# Autodesk Inventor assembly: x_chain_angle
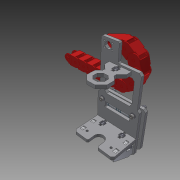
[picture p0: Inventor's stored thumbnail of the model, 180x180]
Saved by Autodesk Inventor 2014 (Build 180170000, 170)
## iProperties
Created: 2013-12-06
Part Number: x_chain_angle
Document SubType Name: Assembly
Designer: buben
Author: buben
## Documents named in this file (4)
- C:\Users\buben\Documents\GitHub\bacon\inventor files\assemblies\x_chain_angle.iam
- C:\Users\buben\Documents\GitHub\bacon\inventor files\assemblies\x_carryage.iam
- C:\Users\buben\Documents\GitHub\bacon\inventor files\utils\x_axis_cable_mount_b.ipt
- C:\Users\buben\Documents\GitHub\bacon\inventor files\utils\cable_chain_22.ipt
## Components (12 placed, 3 different names)
1. x_carryage:1 [sub-assembly] — Flush:1, Mate:1, Mate:2, Mate:3, Mate:4, Mate:5
2. x_axis_cable_mount_b:1 — Mate:3, Mate:4, Mate:5, Insert:10, Mate:6
3. cable_chain_22:1 — Insert:2, Insert:3, Mate:13, Mate:14
4. cable_chain_22:2 — Insert:4, Insert:5, Mate:11, Mate:12
5. cable_chain_22:3 — Insert:1, Mate:15
6. cable_chain_22:4 — Insert:1, Insert:2, Mate:14, Mate:15
7. cable_chain_22:5 — Insert:3, Insert:4, Mate:12, Mate:13
8. cable_chain_22:6 — Insert:5, Insert:6, Mate:10, Mate:11
9. cable_chain_22:7 — Insert:6, Insert:7, Mate:9, Mate:10
10. cable_chain_22:8 — Insert:7, Insert:8, Mate:8, Mate:9
11. cable_chain_22:9 — Insert:8, Insert:9, Mate:7, Mate:8
12. cable_chain_22:10 — Insert:9, Insert:10, Mate:6, Mate:7
## Relationships (26: Mate 15, Insert 10, Flush 1)
- Flush:1: x_carryage:1
- Mate:1: x_carryage:1
- Mate:2: x_carryage:1
- Mate:3: x_carryage:1 ↔ x_axis_cable_mount_b:1
- Mate:4: x_carryage:1 ↔ x_axis_cable_mount_b:1
- Mate:5: x_carryage:1 ↔ x_axis_cable_mount_b:1
- Insert:1: cable_chain_22:3 ↔ cable_chain_22:4
- Insert:2: cable_chain_22:1 ↔ cable_chain_22:4
- Insert:3: cable_chain_22:1 ↔ cable_chain_22:5
- Insert:4: cable_chain_22:2 ↔ cable_chain_22:5
- Insert:5: cable_chain_22:2 ↔ cable_chain_22:6
- Insert:6: cable_chain_22:6 ↔ cable_chain_22:7
- Insert:7: cable_chain_22:7 ↔ cable_chain_22:8
- Insert:8: cable_chain_22:8 ↔ cable_chain_22:9
- Insert:9: cable_chain_22:9 ↔ cable_chain_22:10
- Insert:10: x_axis_cable_mount_b:1 ↔ cable_chain_22:10
- Mate:6: x_axis_cable_mount_b:1 ↔ cable_chain_22:10
- Mate:7: cable_chain_22:9 ↔ cable_chain_22:10
- Mate:8: cable_chain_22:8 ↔ cable_chain_22:9
- Mate:9: cable_chain_22:7 ↔ cable_chain_22:8
- Mate:10: cable_chain_22:6 ↔ cable_chain_22:7
- Mate:11: cable_chain_22:2 ↔ cable_chain_22:6
- Mate:12: cable_chain_22:2 ↔ cable_chain_22:5
- Mate:13: cable_chain_22:1 ↔ cable_chain_22:5
- Mate:14: cable_chain_22:1 ↔ cable_chain_22:4
- Mate:15: cable_chain_22:3 ↔ cable_chain_22:4
